# Autodesk Inventor assembly: Functioning elevator (shaft2)
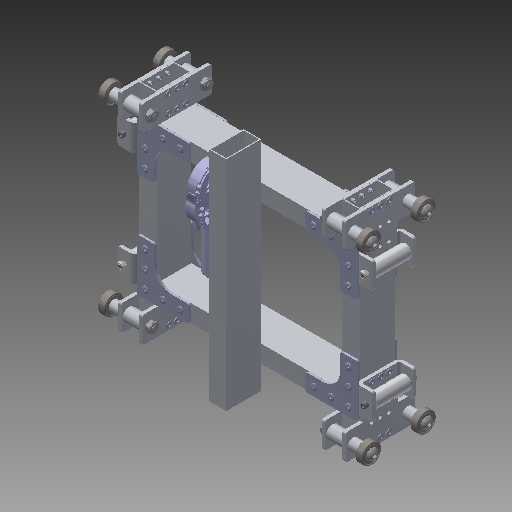
[picture p0: Inventor's stored thumbnail of the model, 512x512]
Saved by Autodesk Inventor 2019 (Build 230136000, 136)
## iProperties
Created: 2019-01-18
Part Number: Functioning elevator (shaft2)
Document SubType Name: Assembly
Designer: josh
Mass: 2149.37 g
Surface Area: 6765.84 cm^2
Volume: 796.062 cm^3
Density: 2.7 g/cm^3
Author: josh
## Documents named in this file (7)
- D:\Synthesis Robots\Epsilon\Epsilon elavator lift\Functioning elevator (shaft2).iam
- D:\Synthesis Robots\Epsilon\Epsilon elavator lift\Functioning elevator parts\Example Bearing Tube.ipt
- D:\Synthesis Robots\Epsilon\Epsilon elavator lift\Functioning elevator parts\Example Single Corner Bearing Assembly R2.iam
- D:\Synthesis Robots\Epsilon\Epsilon elavator lift\Functioning elevator parts\am-3860 90 Gusset with Rivets.iam
- D:\Synthesis Robots\Epsilon\Epsilon elavator lift\Functioning elevator parts\Example Cross Carriage Tube - Copy.ipt
- D:\Synthesis Robots\Epsilon\Epsilon elavator lift\Functioning elevator parts\Bosh motor mount.ipt
- D:\Synthesis Robots\Epsilon\Epsilon Grabbers\FRC Bosch motor V2 6 004 RA3 194-06.ipt
## Components (18 placed, 6 different names)
1. Example Bearing Tube:1 — Mate:22, Mate:24, Mate:25, Mate:26, Flush:11, Flush:12, Flush:13, Flush:15, Mate:30, Mate:31, Mate:32, Mate:33, Mate:40
2. Example Bearing Tube:2 — Flush:3, Flush:4, Mate:3, Mate:4, Mate:5, Mate:7, Mate:8, Mate:9, Mate:10, Mate:11, Mate:12, Flush:5, Flush:6, Flush:8, Mate:17, Mate:19, Mate:34, Mate:38
3. Example Single Corner Bearing Assembly R2:1 [sub-assembly] — Mate:24, Mate:25, Mate:26, Mate:36
4. Example Single Corner Bearing Assembly R2:2 [sub-assembly] — Mate:30, Mate:31, Mate:32, Mate:41
5. Example Single Corner Bearing Assembly R2:3 [sub-assembly] — Mate:10, Mate:11, Mate:12, Mate:13, Mate:14, Mate:16
6. Example Single Corner Bearing Assembly R2:4 [sub-assembly] — Mate:7, Mate:8, Mate:9
7. am-3860 90 Gusset with Rivets:1 [sub-assembly] — Flush:13, Flush:19, Mate:39
8. am-3860 90 Gusset with Rivets:2 [sub-assembly] — Flush:15, Flush:18, Mate:37, Mate:40, Mate:41
9. am-3860 90 Gusset with Rivets:3 [sub-assembly] — Flush:4
10. am-3860 90 Gusset with Rivets:4 [sub-assembly] — Flush:6, Mate:14, Mate:19, Flush:17, Mate:35
11. am-3860 90 Gusset with Rivets:5 [sub-assembly] — Mate:22, Flush:11, Flush:16, Mate:36
12. am-3860 90 Gusset with Rivets:6 [sub-assembly] — Flush:12, Flush:20, Mate:43
13. am-3860 90 Gusset with Rivets:7 [sub-assembly] — Flush:5, Mate:13, Flush:8, Mate:16, Mate:17
14. am-3860 90 Gusset with Rivets:8 [sub-assembly] — Flush:3, Mate:3, Mate:4, Mate:5, Mate:42, Mate:45
15. Example Cross Carriage Tube - Copy:1 — Flush:18, Mate:37, Mate:38, Flush:19, Mate:39, Mate:42, Mate:44
16. Example Cross Carriage Tube - Copy:2 — Mate:33, Flush:16, Flush:17, Mate:34, Mate:35, Flush:20, Mate:43
17. Bosh motor mount:1 — Mate:44, Mate:45, Mate:46, Mate:47
18. FRC Bosch motor V2 6 004 RA3 194-06:1 — Mate:46, Mate:47
## Relationships (50: Mate 36, Flush 14)
- Flush:3: Example Bearing Tube:2 ↔ am-3860 90 Gusset with Rivets:8
- Flush:4: Example Bearing Tube:2 ↔ am-3860 90 Gusset with Rivets:3
- Mate:3: Example Bearing Tube:2 ↔ am-3860 90 Gusset with Rivets:8
- Mate:4: Example Bearing Tube:2 ↔ am-3860 90 Gusset with Rivets:8
- Mate:5: Example Bearing Tube:2 ↔ am-3860 90 Gusset with Rivets:8
- Mate:7: Example Bearing Tube:2 ↔ Example Single Corner Bearing Assembly R2:4
- Mate:8: Example Bearing Tube:2 ↔ Example Single Corner Bearing Assembly R2:4
- Mate:9: Example Bearing Tube:2 ↔ Example Single Corner Bearing Assembly R2:4
- Mate:10: Example Bearing Tube:2 ↔ Example Single Corner Bearing Assembly R2:3
- Mate:11: Example Bearing Tube:2 ↔ Example Single Corner Bearing Assembly R2:3
- Mate:12: Example Bearing Tube:2 ↔ Example Single Corner Bearing Assembly R2:3
- Flush:5: Example Bearing Tube:2 ↔ am-3860 90 Gusset with Rivets:7
- Flush:6: Example Bearing Tube:2 ↔ am-3860 90 Gusset with Rivets:4
- Mate:13: Example Single Corner Bearing Assembly R2:3 ↔ am-3860 90 Gusset with Rivets:7
- Mate:14: Example Single Corner Bearing Assembly R2:3 ↔ am-3860 90 Gusset with Rivets:4
- Flush:8: Example Bearing Tube:2 ↔ am-3860 90 Gusset with Rivets:7
- Mate:16: Example Single Corner Bearing Assembly R2:3 ↔ am-3860 90 Gusset with Rivets:7
- Mate:17: Example Bearing Tube:2 ↔ am-3860 90 Gusset with Rivets:7
- Mate:19: Example Bearing Tube:2 ↔ am-3860 90 Gusset with Rivets:4
- Mate:22: Example Bearing Tube:1 ↔ am-3860 90 Gusset with Rivets:5
- Mate:24: Example Bearing Tube:1 ↔ Example Single Corner Bearing Assembly R2:1
- Mate:25: Example Bearing Tube:1 ↔ Example Single Corner Bearing Assembly R2:1
- Mate:26: Example Bearing Tube:1 ↔ Example Single Corner Bearing Assembly R2:1
- Flush:11: Example Bearing Tube:1 ↔ am-3860 90 Gusset with Rivets:5
- Flush:12: Example Bearing Tube:1 ↔ am-3860 90 Gusset with Rivets:6
- Flush:13: Example Bearing Tube:1 ↔ am-3860 90 Gusset with Rivets:1
- Flush:15: Example Bearing Tube:1 ↔ am-3860 90 Gusset with Rivets:2
- Mate:30: Example Bearing Tube:1 ↔ Example Single Corner Bearing Assembly R2:2
- Mate:31: Example Bearing Tube:1 ↔ Example Single Corner Bearing Assembly R2:2
- Mate:32: Example Bearing Tube:1 ↔ Example Single Corner Bearing Assembly R2:2
- Mate:33: Example Bearing Tube:1 ↔ Example Cross Carriage Tube - Copy:2
- Flush:16: am-3860 90 Gusset with Rivets:5 ↔ Example Cross Carriage Tube - Copy:2
- Flush:17: am-3860 90 Gusset with Rivets:4 ↔ Example Cross Carriage Tube - Copy:2
- Mate:34: Example Bearing Tube:2 ↔ Example Cross Carriage Tube - Copy:2
- Mate:35: am-3860 90 Gusset with Rivets:4 ↔ Example Cross Carriage Tube - Copy:2
- Mate:36: Example Single Corner Bearing Assembly R2:1 ↔ am-3860 90 Gusset with Rivets:5
- Flush:18: am-3860 90 Gusset with Rivets:2 ↔ Example Cross Carriage Tube - Copy:1
- Mate:37: am-3860 90 Gusset with Rivets:2 ↔ Example Cross Carriage Tube - Copy:1
- Mate:38: Example Bearing Tube:2 ↔ Example Cross Carriage Tube - Copy:1
- Flush:19: am-3860 90 Gusset with Rivets:1 ↔ Example Cross Carriage Tube - Copy:1
- Mate:39: am-3860 90 Gusset with Rivets:1 ↔ Example Cross Carriage Tube - Copy:1
- Mate:40: Example Bearing Tube:1 ↔ am-3860 90 Gusset with Rivets:2
- Mate:41: Example Single Corner Bearing Assembly R2:2 ↔ am-3860 90 Gusset with Rivets:2
- Mate:42: am-3860 90 Gusset with Rivets:8 ↔ Example Cross Carriage Tube - Copy:1
- Flush:20: am-3860 90 Gusset with Rivets:6 ↔ Example Cross Carriage Tube - Copy:2
- Mate:43: am-3860 90 Gusset with Rivets:6 ↔ Example Cross Carriage Tube - Copy:2
- Mate:44: Example Cross Carriage Tube - Copy:1 ↔ Bosh motor mount:1
- Mate:45 (67.3354 mm): am-3860 90 Gusset with Rivets:8 ↔ Bosh motor mount:1
- Mate:46: Bosh motor mount:1 ↔ FRC Bosch motor V2 6 004 RA3 194-06:1
- Mate:47 (12.7 mm): Bosh motor mount:1 ↔ FRC Bosch motor V2 6 004 RA3 194-06:1
